# Autodesk Inventor assembly: Arm Assembly
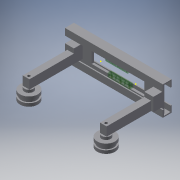
[picture p0: Inventor's stored thumbnail of the model, 180x180]
Saved by Autodesk Inventor 2017 (Build 210142000, 142)
## iProperties
Created: 2017-10-11
Part Number: Arm Assembly
Document SubType Name: Assembly
Designer: Kenneth
Author: Kenneth
## Documents named in this file (7)
- C:\Workspaces\CAD\Arm Parts\Arm Assembly.iam
- C:\Workspaces\CAD\Arm Parts\Back Slide plate.ipt
- C:\Workspaces\CAD\Arm Parts\Back slide plate and side bar attatchment.ipt
- C:\Workspaces\CAD\Arm Parts\Side Bar.ipt
- C:\Workspaces\CAD\Spectrum-CAD-Library\Vex EDR\Gears\Rack Gear.ipt
- C:\Workspaces\CAD\Arm Parts\Pulley.ipt
- C:\Workspaces\CAD\Arm Parts\case.ipt
## Components (12 placed, 6 different names)
1. Back Slide plate:1 — Flush:1, Flush:2, Mate:3, Flush:6, Flush:12, Mate:11, Flush:18, Mate:16, Mate:17, Mate:20, Mate:22
2. Back Slide plate:2 — Flush:1, Flush:2, Mate:2, Flush:4, Flush:13, Mate:12, Flush:16, Mate:18, Mate:19, Mate:21, Mate:23
3. Back slide plate and side bar attatchment:1 — Mate:3, Flush:6, Mate:4, Flush:10, Mate:17, Flush:20, Mate:20
4. Back slide plate and side bar attatchment:2 — Mate:2, Flush:4, Mate:5, Flush:9, Mate:18, Flush:19, Mate:19
5. Side Bar:1 — Mate:5, Flush:9, Flush:19, Mate:26, Mate:27
6. Side Bar:2 — Mate:4, Flush:10, Flush:20, Mate:24, Mate:25
7. Rack Gear:1 — Flush:12, Mate:11, Flush:18
8. Rack Gear:4 — Flush:13, Mate:12, Flush:16
9. Pulley:2 — Mate:26, Mate:27
10. Pulley:3 — Mate:24, Mate:25
11. case:1 — Mate:16, Mate:23, Flush:21
12. case:2 — Mate:21, Mate:22, Flush:21
## Relationships (31: Mate 18, Flush 13)
- Flush:1: Back Slide plate:1 ↔ Back Slide plate:2
- Flush:2 (6.35 mm): Back Slide plate:1 ↔ Back Slide plate:2
- Mate:2: Back Slide plate:2 ↔ Back slide plate and side bar attatchment:2
- Flush:4: Back Slide plate:2 ↔ Back slide plate and side bar attatchment:2
- Mate:3: Back Slide plate:1 ↔ Back slide plate and side bar attatchment:1
- Flush:6: Back Slide plate:1 ↔ Back slide plate and side bar attatchment:1
- Mate:4: Back slide plate and side bar attatchment:1 ↔ Side Bar:2
- Mate:5: Back slide plate and side bar attatchment:2 ↔ Side Bar:1
- Flush:9: Back slide plate and side bar attatchment:2 ↔ Side Bar:1
- Flush:10: Back slide plate and side bar attatchment:1 ↔ Side Bar:2
- Flush:12: Back Slide plate:1 ↔ Rack Gear:1
- Mate:11: Back Slide plate:1 ↔ Rack Gear:1
- Flush:13: Back Slide plate:2 ↔ Rack Gear:4
- Mate:12: Back Slide plate:2 ↔ Rack Gear:4
- Flush:16: Back Slide plate:2 ↔ Rack Gear:4
- Flush:18: Back Slide plate:1 ↔ Rack Gear:1
- Mate:16: Back Slide plate:1 ↔ case:1
- Mate:17: Back Slide plate:1 ↔ Back slide plate and side bar attatchment:1
- Mate:18: Back Slide plate:2 ↔ Back slide plate and side bar attatchment:2
- Flush:19: Back slide plate and side bar attatchment:2 ↔ Side Bar:1
- Flush:20: Back slide plate and side bar attatchment:1 ↔ Side Bar:2
- Mate:19: Back Slide plate:2 ↔ Back slide plate and side bar attatchment:2
- Mate:20: Back Slide plate:1 ↔ Back slide plate and side bar attatchment:1
- Mate:21: Back Slide plate:2 ↔ case:2
- Mate:22: Back Slide plate:1 ↔ case:2
- Mate:23: Back Slide plate:2 ↔ case:1
- Mate:24: Side Bar:2 ↔ Pulley:3
- Mate:25: Side Bar:2 ↔ Pulley:3
- Mate:26: Side Bar:1 ↔ Pulley:2
- Mate:27: Side Bar:1 ↔ Pulley:2
- Flush:21: case:1 ↔ case:2
